# Autodesk Inventor assembly: 自動販賣機3.4
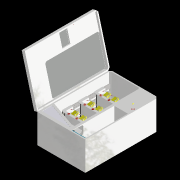
[picture p0: Inventor's stored thumbnail of the model, 180x180]
Saved by Autodesk Inventor 2020 (Build 240168000, 168)
## iProperties
Created: 2021-04-08
Part Number: 自動販賣機3.4
Document SubType Name: Assembly
Designer: 88690
Author: 88690
## Documents named in this file (33)
- C:\Users\88690\Desktop\自動販賣機\自動販賣機3.4.iam
- C:\Users\88690\Desktop\自動販賣機\上滑軌.ipt
- C:\Users\88690\Desktop\自動販賣機\上滑軌輪.ipt
- C:\Users\88690\Desktop\自動販賣機\下滑軌.ipt
- C:\Users\88690\Desktop\自動販賣機\下滑軌輪.ipt
- C:\Users\88690\Desktop\自動販賣機\本體.ipt
- C:\Users\88690\Desktop\自動販賣機\置物架.ipt
- C:\Users\88690\Desktop\自動販賣機\滾筒.ipt
- C:\Users\88690\Desktop\自動販賣機\蓋.ipt
- C:\Users\88690\Desktop\自動販賣機\鎖點支架.ipt
- C:\Users\88690\Desktop\自動販賣機\下支架右.ipt
- C:\Users\88690\Desktop\自動販賣機\上滑軌右.ipt
- C:\Users\88690\Desktop\自動販賣機\蝸桿支架.ipt
- C:\Users\88690\Desktop\自動販賣機\蝸桿滑塊.ipt
- C:\Users\88690\Desktop\自動販賣機\短蝸桿.ipt
- C:\Users\88690\Desktop\自動販賣機\長蝸桿.ipt
- C:\Users\88690\Desktop\自動販賣機\位移平台.ipt
- C:\Users\88690\Desktop\自動販賣機\取物窗.ipt
- C:\Users\88690\Desktop\自動販賣機\螺旋鉤子.ipt
- C:\Users\88690\Desktop\自動販賣機\螺旋鉤子底座.ipt
- C:\Users\88690\Desktop\自動販賣機\名牌1.ipt
- C:\Users\88690\Desktop\自動販賣機\名牌2.ipt
- C:\Users\88690\Desktop\自動販賣機\模擬商品.ipt
- C:\Users\88690\Desktop\自動販賣機\模擬錢幣.ipt
- C:\Users\88690\Desktop\自動販賣機\商品支架.ipt
- C:\Users\88690\Desktop\自動販賣機\名牌3.ipt
- C:\Users\88690\Desktop\自動販賣機\名牌4.ipt
- C:\Users\88690\Desktop\自動販賣機\名牌5.ipt
- C:\Users\88690\Desktop\自動販賣機\名牌6.ipt
- C:\Users\88690\Desktop\自動販賣機\名牌7.ipt
- C:\Users\88690\Desktop\自動販賣機\名牌8.ipt
- C:\Users\88690\Desktop\自動販賣機\名牌9.ipt
- C:\Users\88690\Desktop\自動販賣機\玻璃窗.ipt
## Components (110 placed, 32 different names)
1. 上滑軌:1 — 貼合:41, 貼合:42, 貼合:45, 相切:7, 貼合:183
2. 上滑軌輪:1 — 貼合:41, 貼合:42, 相切:1
3. 下滑軌:1 — 貼合:11, 貼合:12, 貼合:13, 貼合:15, 相切:1, 角度:40
4. 下滑軌輪:1 — 貼合:11, 貼合:12, 相切:7
5. 本體:1 — 齊平:1, 齊平:2, 齊平:3, 貼合:1, 貼合:2, 貼合:3, 貼合:4, 貼合:6, 貼合:7, 貼合:8, 貼合:9, 貼合:75, 貼合:76, 貼合:77, 貼合:78, 貼合:79, 貼合:80, 貼合:81, 貼合:82, 貼合:83, 貼合:84, 貼合:85, 貼合:86, 貼合:88, 貼合:89, 貼合:101, 齊平:23, 角度:1, 旋轉:1, 貼合:167, 角度:34, 貼合:169, 貼合:171, 貼合:172, 齊平:53, 齊平:58, 齊平:69
6. 置物架:1 — 貼合:45, 貼合:50, 貼合:51, 貼合:131, 貼合:143, 貼合:144, 貼合:145, 旋轉:3, 齊平:53, 角度:40, 貼合:183, 角度:41, 貼合:187, 相切:13, 相切:15, 貼合:227, 貼合:228, 貼合:229, 相切:16, 貼合:298, 貼合:299, 相切:17, 相切:18, 相切:19, 貼合:300, 貼合:301, 相切:20, 相切:21, 相切:22, 齊平:66, 齊平:67, 齊平:68, 貼合:448
7. 滾筒:1 — 貼合:75, 貼合:76, 齊平:14, 齊平:15, 齊平:16, 齊平:17, 齊平:18, 齊平:19, 齊平:20, 齊平:21, 齊平:22, 角度:12, 旋轉:1, 旋轉:1
8. 蓋:1 — 貼合:101, 齊平:23, 角度:1, 角度:2, 貼合:108, 貼合:164, 角度:34, 角度:35, 齊平:78, 貼合:455, 貼合:456
9. 鎖點支架:1 — 貼合:1, 貼合:2, 貼合:3, 齊平:4, 齊平:5, 齊平:6, 齊平:7, 貼合:5, 貼合:15
10. 鎖點支架:2 — 齊平:5, 齊平:7, 貼合:5, 貼合:13, 貼合:51
11. 鎖點支架:3 — 齊平:4, 齊平:6, 貼合:4
12. 鎖點支架:4 — 齊平:8, 齊平:10, 貼合:9
13. 鎖點支架:5 — 貼合:6, 貼合:7, 貼合:8, 齊平:8, 齊平:9, 齊平:10, 齊平:11, 貼合:10, 貼合:30
14. 鎖點支架:6 — 齊平:9, 齊平:11, 貼合:10, 貼合:28
15. 下支架右:1 — 貼合:26, 貼合:27, 貼合:28, 貼合:30, 相切:2, 貼合:74, 角度:41
16. 下滑軌輪:4 — 貼合:26, 貼合:27, 相切:10
17. 上滑軌右:1 — 貼合:46, 貼合:50, 相切:10, 貼合:186, 貼合:187
18. 上滑軌輪:2 — 貼合:46, 相切:2, 貼合:74, 貼合:186
19. 滾筒:2 — 齊平:14, 貼合:77, 旋轉:1, 旋轉:2, 角度:13
20. 滾筒:3 — 齊平:15, 貼合:78, 旋轉:2, 角度:14, 旋轉:3
21. 滾筒:4 — 齊平:16, 貼合:79, 角度:15, 旋轉:3, 旋轉:4
22. 滾筒:5 — 齊平:17, 貼合:80, 角度:16, 旋轉:4, 旋轉:5
23. 滾筒:6 — 齊平:18, 貼合:81, 角度:18, 旋轉:5, 旋轉:6
24. 滾筒:7 — 齊平:19, 貼合:82, 角度:19, 旋轉:6, 旋轉:7
25. 滾筒:8 — 齊平:20, 貼合:83, 角度:22, 旋轉:7, 旋轉:8
26. 滾筒:9 — 齊平:21, 貼合:84, 角度:20, 旋轉:8, 旋轉:9
27. 滾筒:10 — 齊平:22, 貼合:85, 角度:21, 旋轉:9
28. 蝸桿支架:1 — 貼合:86, 貼合:88, 貼合:89, 貼合:90, 貼合:91, 貼合:92, 貼合:93
29. 蝸桿滑塊:1 — 貼合:90, 貼合:91, 貼合:94, 貼合:95, 貼合:97, 貼合:98, 貼合:99
30. 短蝸桿:1 — 貼合:94, 貼合:95, 旋轉/轉換:1
31. 長蝸桿:1 — 貼合:92, 貼合:93, 角度:23, 旋轉/轉換:1
32. 位移平台:1 — 貼合:97, 貼合:98, 貼合:99, 貼合:167
33. 取物窗:1 — 角度:2, 貼合:108, 貼合:164, 角度:35
34. 螺旋鉤子:2 — 貼合:131, 角度:45, 貼合:221, 貼合:223, 貼合:230, 貼合:231, 貼合:232, 貼合:233
35. 螺旋鉤子底座:2 — 旋轉:3, 角度:44
36. 名牌1:1 — 貼合:143, 貼合:144, 角度:24, 齊平:30, 角度:25
37. 名牌2:1 — 貼合:145, 齊平:30, 角度:25, 齊平:71, 齊平:72, 角度:52
38. 模擬錢幣:1 — 貼合:169, 貼合:171, 貼合:172
39. 模擬商品:2 — 貼合:221, 相切:13, 貼合:230
40. 商品支架:1 — 貼合:227, 貼合:228, 貼合:229
41. 模擬商品:22 — 貼合:223, 相切:15, 貼合:231
42. 模擬商品:23 — 相切:16, 貼合:232, 貼合:233
43. 螺旋鉤子:3
44. 螺旋鉤子底座:3 — 貼合:298, 貼合:299
45. 模擬商品:24 — 相切:17
46. 模擬商品:25 — 相切:18
47. 模擬商品:26 — 相切:19
48. 螺旋鉤子:4
49. 螺旋鉤子底座:4 — 貼合:300, 貼合:301
50. 模擬商品:27 — 相切:20
51. 模擬商品:28 — 相切:21
52. 模擬商品:29 — 相切:22
53. 上滑軌:2 — 齊平:57
54. 上滑軌輪:3 — 貼合:398
55. 下滑軌:2 — 齊平:60, 貼合:398
56. 下滑軌輪:5
57. 置物架:2 — 齊平:56, 齊平:58, 齊平:59, 齊平:60, 齊平:66, 齊平:67, 齊平:70, 貼合:449, 貼合:450, 貼合:451
58. 下支架右:2 — 齊平:59
59. 下滑軌輪:6
60. 上滑軌右:2 — 齊平:56, 齊平:57
61. 上滑軌輪:4
62. 螺旋鉤子:5
63. 螺旋鉤子底座:5
64. 模擬商品:30
65. 商品支架:2
66. 模擬商品:31
67. 模擬商品:32
68. 螺旋鉤子:6
69. 螺旋鉤子底座:6
70. 模擬商品:33
71. 模擬商品:34
72. 模擬商品:35
73. 螺旋鉤子:7
74. 螺旋鉤子底座:7
75. 模擬商品:36
76. 模擬商品:37
77. 模擬商品:38
78. 上滑軌:3
79. 上滑軌輪:5
80. 下滑軌:3
81. 下滑軌輪:7
82. 置物架:3 — 齊平:68, 齊平:69, 齊平:70, 貼合:452, 貼合:453, 貼合:454
83. 下支架右:3
84. 下滑軌輪:8
85. 上滑軌右:3
86. 上滑軌輪:6
87. 螺旋鉤子:8
88. 螺旋鉤子底座:8
89. 模擬商品:39
90. 商品支架:3
91. 模擬商品:40
92. 模擬商品:41
93. 螺旋鉤子:9
94. 螺旋鉤子底座:9
95. 模擬商品:42
96. 模擬商品:43
97. 模擬商品:44
98. 螺旋鉤子:10
99. 螺旋鉤子底座:10
100. 模擬商品:45
101. 模擬商品:46
102. 模擬商品:47
103. 名牌3:1 — 貼合:448, 齊平:71, 角度:52, 角度:53
104. 名牌4:1 — 貼合:449, 齊平:72, 齊平:73, 角度:53, 角度:54
105. 名牌5:1 — 貼合:450, 齊平:73, 齊平:74, 角度:54, 角度:55
106. 名牌6:1 — 貼合:451, 齊平:74, 齊平:75, 角度:55, 角度:56
107. 名牌7:1 — 貼合:452, 齊平:77, 角度:56, 角度:57
108. 名牌8:1 — 貼合:453, 齊平:76, 齊平:77, 角度:57, 角度:58
109. 名牌9:1 — 貼合:454, 齊平:75, 齊平:76, 角度:58
110. 玻璃窗:1 — 齊平:78, 貼合:455, 貼合:456
## Relationships (324: Mate 194, Flush 45, Tangent 39, Angle 32, RelateRotation 9, RevoluteJoint 4, RelateRotateTranslate 1)
- 齊平:1 [Flush]: 本體:1
- 齊平:2 [Flush]: 本體:1
- 齊平:3 [Flush]: 本體:1
- 貼合:1 [Mate] (180 mm): 本體:1 ↔ 鎖點支架:1
- 貼合:2 [Mate]: 本體:1 ↔ 鎖點支架:1
- 貼合:3 [Mate]: 本體:1 ↔ 鎖點支架:1
- 齊平:4 [Flush]: 鎖點支架:1 ↔ 鎖點支架:3
- 齊平:5 [Flush]: 鎖點支架:1 ↔ 鎖點支架:2
- 齊平:6 [Flush]: 鎖點支架:1 ↔ 鎖點支架:3
- 齊平:7 [Flush]: 鎖點支架:1 ↔ 鎖點支架:2
- 貼合:4 [Mate]: 本體:1 ↔ 鎖點支架:3
- 貼合:5 [Mate] (55 mm): 鎖點支架:1 ↔ 鎖點支架:2
- 貼合:6 [Mate]: 本體:1 ↔ 鎖點支架:5
- 貼合:7 [Mate]: 本體:1 ↔ 鎖點支架:5
- 貼合:8 [Mate] (180 mm): 本體:1 ↔ 鎖點支架:5
- 齊平:8 [Flush]: 鎖點支架:4 ↔ 鎖點支架:5
- 齊平:9 [Flush]: 鎖點支架:5 ↔ 鎖點支架:6
- 齊平:10 [Flush]: 鎖點支架:4 ↔ 鎖點支架:5
- 齊平:11 [Flush]: 鎖點支架:5 ↔ 鎖點支架:6
- 貼合:9 [Mate]: 本體:1 ↔ 鎖點支架:4
- 貼合:10 [Mate] (55 mm): 鎖點支架:5 ↔ 鎖點支架:6
- 貼合:11 [Mate]: 下滑軌:1 ↔ 下滑軌輪:1
- 貼合:12 [Mate]: 下滑軌:1 ↔ 下滑軌輪:1
- 貼合:13 [Mate]: 下滑軌:1 ↔ 鎖點支架:2
- 貼合:15 [Mate]: 下滑軌:1 ↔ 鎖點支架:1
- 貼合:26 [Mate]: 下支架右:1 ↔ 下滑軌輪:4
- 貼合:27 [Mate]: 下支架右:1 ↔ 下滑軌輪:4
- 貼合:28 [Mate]: 鎖點支架:6 ↔ 下支架右:1
- 貼合:30 [Mate]: 鎖點支架:5 ↔ 下支架右:1
- 貼合:41 [Mate]: 上滑軌:1 ↔ 上滑軌輪:1
- 貼合:42 [Mate]: 上滑軌:1 ↔ 上滑軌輪:1
- 貼合:45 [Mate]: 上滑軌:1 ↔ 置物架:1
- 貼合:46 [Mate]: 上滑軌右:1 ↔ 上滑軌輪:2
- 貼合:50 [Mate]: 置物架:1 ↔ 上滑軌右:1
- 相切:1 [Tangent]: 上滑軌輪:1 ↔ 下滑軌:1
- 相切:2 [Tangent]: 下支架右:1 ↔ 上滑軌輪:2
- 貼合:51 [Mate]: 置物架:1 ↔ 鎖點支架:2
- 貼合:74 [Mate]: 下支架右:1 ↔ 上滑軌輪:2
- 貼合:75 [Mate]: 本體:1 ↔ 滾筒:1
- 貼合:76 [Mate]: 本體:1 ↔ 滾筒:1
- 齊平:14 [Flush]: 滾筒:1 ↔ 滾筒:2
- 齊平:15 [Flush]: 滾筒:1 ↔ 滾筒:3
- 齊平:16 [Flush]: 滾筒:1 ↔ 滾筒:4
- 齊平:17 [Flush]: 滾筒:1 ↔ 滾筒:5
- 齊平:18 [Flush]: 滾筒:1 ↔ 滾筒:6
- 齊平:19 [Flush]: 滾筒:1 ↔ 滾筒:7
- 齊平:20 [Flush]: 滾筒:1 ↔ 滾筒:8
- 齊平:21 [Flush]: 滾筒:1 ↔ 滾筒:9
- 齊平:22 [Flush]: 滾筒:1 ↔ 滾筒:10
- 貼合:77 [Mate]: 本體:1 ↔ 滾筒:2
- 貼合:78 [Mate]: 本體:1 ↔ 滾筒:3
- 貼合:79 [Mate]: 本體:1 ↔ 滾筒:4
- 貼合:80 [Mate]: 本體:1 ↔ 滾筒:5
- 貼合:81 [Mate]: 本體:1 ↔ 滾筒:6
- 貼合:82 [Mate]: 本體:1 ↔ 滾筒:7
- 貼合:83 [Mate]: 本體:1 ↔ 滾筒:8
- 貼合:84 [Mate]: 本體:1 ↔ 滾筒:9
- 貼合:85 [Mate]: 本體:1 ↔ 滾筒:10
- 貼合:86 [Mate]: 本體:1 ↔ 蝸桿支架:1
- 貼合:88 [Mate]: 本體:1 ↔ 蝸桿支架:1
- 貼合:89 [Mate]: 本體:1 ↔ 蝸桿支架:1
- 貼合:90 [Mate]: 蝸桿支架:1 ↔ 蝸桿滑塊:1
- 貼合:91 [Mate]: 蝸桿支架:1 ↔ 蝸桿滑塊:1
- 貼合:92 [Mate]: 蝸桿支架:1 ↔ 長蝸桿:1
- 貼合:93 [Mate]: 蝸桿支架:1 ↔ 長蝸桿:1
- 貼合:94 [Mate]: 蝸桿滑塊:1 ↔ 短蝸桿:1
- 貼合:95 [Mate]: 蝸桿滑塊:1 ↔ 短蝸桿:1
- 貼合:97 [Mate]: 蝸桿滑塊:1 ↔ 位移平台:1
- 貼合:98 [Mate]: 蝸桿滑塊:1 ↔ 位移平台:1
- 貼合:99 [Mate]: 蝸桿滑塊:1 ↔ 位移平台:1
- 貼合:101 [Mate]: 本體:1 ↔ 蓋:1
- 齊平:23 [Flush]: 本體:1 ↔ 蓋:1
- 角度:1 [Angle] (45 deg): 本體:1 ↔ 蓋:1
- 角度:2 [Angle] (180 deg): 蓋:1 ↔ 取物窗:1
- 貼合:108 [Mate]: 蓋:1 ↔ 取物窗:1
- [Mate]: 螺旋鉤子:2 ↔ 螺旋鉤子底座:2
- [Mate]: 螺旋鉤子:2 ↔ 螺旋鉤子底座:2
- 貼合:131 [Mate]: 置物架:1 ↔ 螺旋鉤子:2
- 角度:12 [Angle] (4455 deg): 滾筒:1
- 旋轉:1 [RelateRotation] (1 ul): 滾筒:1 ↔ 滾筒:2
- 旋轉:2 [RelateRotation] (1 ul): 滾筒:2 ↔ 滾筒:3
- 角度:13 [Angle] (135 deg): 滾筒:2
- 角度:14 [Angle] (135 deg): 滾筒:3
- 角度:15 [Angle] (135 deg): 滾筒:4
- 角度:16 [Angle] (135 deg): 滾筒:5
- 角度:18 [Angle] (135 deg): 滾筒:6
- 角度:19 [Angle] (135 deg): 滾筒:7
- 角度:20 [Angle] (135 deg): 滾筒:9
- 角度:21 [Angle] (135 deg): 滾筒:10
- 角度:22 [Angle] (135 deg): 滾筒:8
- 旋轉:3 [RelateRotation] (1 ul): 滾筒:3 ↔ 滾筒:4
- 旋轉:4 [RelateRotation] (1 ul): 滾筒:4 ↔ 滾筒:5
- 旋轉:5 [RelateRotation] (1 ul): 滾筒:5 ↔ 滾筒:6
- 旋轉:6 [RelateRotation] (1 ul): 滾筒:6 ↔ 滾筒:7
- 旋轉:7 [RelateRotation] (1 ul): 滾筒:7 ↔ 滾筒:8
- 旋轉:8 [RelateRotation] (1 ul): 滾筒:8 ↔ 滾筒:9
- 旋轉:9 [RelateRotation] (1 ul): 滾筒:9 ↔ 滾筒:10
- 旋轉:1 [RevoluteJoint]: 本體:1 ↔ 滾筒:1
- 角度:23 [Angle] (0 deg): 長蝸桿:1
- 旋轉/轉換:1 [RelateRotateTranslate] (103.673 mm): 短蝸桿:1 ↔ 長蝸桿:1
- 貼合:143 [Mate]: 置物架:1 ↔ 名牌1:1
- 貼合:144 [Mate]: 置物架:1 ↔ 名牌1:1
- 角度:24 [Angle] (0 deg): 名牌1:1
- 貼合:145 [Mate]: 置物架:1 ↔ 名牌2:1
- 齊平:30 [Flush]: 名牌1:1 ↔ 名牌2:1
- 角度:25 [Angle] (0 deg): 名牌1:1 ↔ 名牌2:1
- 旋轉:3 [RevoluteJoint]: 置物架:1 ↔ 螺旋鉤子底座:2
- 貼合:164 [Mate]: 蓋:1 ↔ 取物窗:1
- 貼合:167 [Mate]: 本體:1 ↔ 位移平台:1
- 角度:34 [Angle] (75 deg): 本體:1 ↔ 蓋:1
- 角度:35 [Angle] (180 deg): 蓋:1 ↔ 取物窗:1
- 貼合:169 [Mate] (0.5 mm): 本體:1 ↔ 模擬錢幣:1
- 貼合:171 [Mate]: 本體:1 ↔ 模擬錢幣:1
- 貼合:172 [Mate] (150 mm): 本體:1 ↔ 模擬錢幣:1
- 齊平:53 [Flush] (-390 mm): 本體:1 ↔ 置物架:1
- 角度:40 [Angle] (0 deg): 下滑軌:1 ↔ 置物架:1
- 相切:7 [Tangent]: 上滑軌:1 ↔ 下滑軌輪:1
- 貼合:183 [Mate]: 上滑軌:1 ↔ 置物架:1
- 角度:41 [Angle] (0 deg): 置物架:1 ↔ 下支架右:1
- 相切:10 [Tangent]: 下滑軌輪:4 ↔ 上滑軌右:1
- 貼合:186 [Mate]: 上滑軌右:1 ↔ 上滑軌輪:2
- 貼合:187 [Mate]: 置物架:1 ↔ 上滑軌右:1
- 角度:44 [Angle] (0 deg): 螺旋鉤子底座:2
- 角度:45 [Angle] (180 deg): 螺旋鉤子:2
- 貼合:221 [Mate]: 螺旋鉤子:2 ↔ 模擬商品:2
- 相切:13 [Tangent]: 置物架:1 ↔ 模擬商品:2
- 貼合:223 [Mate]: 螺旋鉤子:2 ↔ 模擬商品:22
- 相切:15 [Tangent]: 置物架:1 ↔ 模擬商品:22
- 貼合:227 [Mate]: 置物架:1 ↔ 商品支架:1
- 貼合:228 [Mate]: 置物架:1 ↔ 商品支架:1
- 貼合:229 [Mate]: 置物架:1 ↔ 商品支架:1
- 貼合:230 [Mate]: 螺旋鉤子:2 ↔ 模擬商品:2
- 貼合:231 [Mate]: 螺旋鉤子:2 ↔ 模擬商品:22
- 相切:16 [Tangent]: 置物架:1 ↔ 模擬商品:23
- 貼合:232 [Mate]: 螺旋鉤子:2 ↔ 模擬商品:23
- 貼合:233 [Mate]: 螺旋鉤子:2 ↔ 模擬商品:23
- [Mate]: 螺旋鉤子:3 ↔ 螺旋鉤子底座:3
- [Mate]: 螺旋鉤子:3 ↔ 螺旋鉤子底座:3
- [Mate]: 螺旋鉤子:3 ↔ 模擬商品:24
- [Mate]: 螺旋鉤子:3 ↔ 模擬商品:25
- [Mate]: 螺旋鉤子:3 ↔ 模擬商品:24
- [Mate]: 螺旋鉤子:3 ↔ 模擬商品:25
- [Mate]: 螺旋鉤子:3 ↔ 模擬商品:26
- [Mate]: 螺旋鉤子:3 ↔ 模擬商品:26
- [Mate]: 螺旋鉤子:4 ↔ 螺旋鉤子底座:4
- [Mate]: 螺旋鉤子:4 ↔ 螺旋鉤子底座:4
- [Mate]: 螺旋鉤子:4 ↔ 模擬商品:27
- [Mate]: 螺旋鉤子:4 ↔ 模擬商品:28
- [Mate]: 螺旋鉤子:4 ↔ 模擬商品:27
- [Mate]: 螺旋鉤子:4 ↔ 模擬商品:28
- [Mate]: 螺旋鉤子:4 ↔ 模擬商品:29
- [Mate]: 螺旋鉤子:4 ↔ 模擬商品:29
- 貼合:298 [Mate]: 置物架:1 ↔ 螺旋鉤子底座:3
- 貼合:299 [Mate]: 置物架:1 ↔ 螺旋鉤子底座:3
- 相切:17 [Tangent]: 置物架:1 ↔ 模擬商品:24
- 相切:18 [Tangent]: 置物架:1 ↔ 模擬商品:25
- 相切:19 [Tangent]: 置物架:1 ↔ 模擬商品:26
- 貼合:300 [Mate]: 置物架:1 ↔ 螺旋鉤子底座:4
- 貼合:301 [Mate]: 置物架:1 ↔ 螺旋鉤子底座:4
- 相切:20 [Tangent]: 置物架:1 ↔ 模擬商品:27
- 相切:21 [Tangent]: 置物架:1 ↔ 模擬商品:28
- 相切:22 [Tangent]: 置物架:1 ↔ 模擬商品:29
- [Mate]: 下滑軌:2 ↔ 下滑軌輪:5
- [Mate]: 下滑軌:2 ↔ 下滑軌輪:5
- [Mate]: 下支架右:2 ↔ 下滑軌輪:6
- [Mate]: 下支架右:2 ↔ 下滑軌輪:6
- [Mate]: 上滑軌:2 ↔ 上滑軌輪:3
- [Mate]: 上滑軌:2 ↔ 上滑軌輪:3
- [Mate]: 上滑軌:2 ↔ 置物架:2
- [Mate]: 上滑軌右:2 ↔ 上滑軌輪:4
- [Mate]: 置物架:2 ↔ 上滑軌右:2
- [Tangent]: 上滑軌輪:3 ↔ 下滑軌:2
- [Tangent]: 下支架右:2 ↔ 上滑軌輪:4
- [Mate]: 下支架右:2 ↔ 上滑軌輪:4
- [Mate]: 螺旋鉤子:5 ↔ 螺旋鉤子底座:5
- [Mate]: 螺旋鉤子:5 ↔ 螺旋鉤子底座:5
- [Mate]: 置物架:2 ↔ 螺旋鉤子:5
- [RevoluteJoint]: 置物架:2 ↔ 螺旋鉤子底座:5
- [Angle] (0 deg): 下滑軌:2 ↔ 置物架:2
- [Tangent]: 上滑軌:2 ↔ 下滑軌輪:5
- [Mate]: 上滑軌:2 ↔ 置物架:2
- [Angle] (0 deg): 置物架:2 ↔ 下支架右:2
- [Tangent]: 下滑軌輪:6 ↔ 上滑軌右:2
- [Mate]: 上滑軌右:2 ↔ 上滑軌輪:4
- [Mate]: 置物架:2 ↔ 上滑軌右:2
- [Mate]: 螺旋鉤子:5 ↔ 模擬商品:30
- [Tangent]: 置物架:2 ↔ 模擬商品:30
- [Mate]: 螺旋鉤子:5 ↔ 模擬商品:31
- [Tangent]: 置物架:2 ↔ 模擬商品:31
- [Mate]: 置物架:2 ↔ 商品支架:2
- [Mate]: 置物架:2 ↔ 商品支架:2
- [Mate]: 置物架:2 ↔ 商品支架:2
- [Mate]: 螺旋鉤子:5 ↔ 模擬商品:30
- [Mate]: 螺旋鉤子:5 ↔ 模擬商品:31
- [Tangent]: 置物架:2 ↔ 模擬商品:32
- [Mate]: 螺旋鉤子:5 ↔ 模擬商品:32
- [Mate]: 螺旋鉤子:5 ↔ 模擬商品:32
- [Mate]: 螺旋鉤子:6 ↔ 螺旋鉤子底座:6
- [Mate]: 螺旋鉤子:6 ↔ 螺旋鉤子底座:6
- [Mate]: 螺旋鉤子:6 ↔ 模擬商品:33
- [Mate]: 螺旋鉤子:6 ↔ 模擬商品:34
- [Mate]: 螺旋鉤子:6 ↔ 模擬商品:33
- [Mate]: 螺旋鉤子:6 ↔ 模擬商品:34
- [Mate]: 螺旋鉤子:6 ↔ 模擬商品:35
- [Mate]: 螺旋鉤子:6 ↔ 模擬商品:35
- [Mate]: 螺旋鉤子:7 ↔ 螺旋鉤子底座:7
- [Mate]: 螺旋鉤子:7 ↔ 螺旋鉤子底座:7
- [Mate]: 螺旋鉤子:7 ↔ 模擬商品:36
- [Mate]: 螺旋鉤子:7 ↔ 模擬商品:37
- [Mate]: 螺旋鉤子:7 ↔ 模擬商品:36
- [Mate]: 螺旋鉤子:7 ↔ 模擬商品:37
- [Mate]: 螺旋鉤子:7 ↔ 模擬商品:38
- [Mate]: 螺旋鉤子:7 ↔ 模擬商品:38
- [Mate]: 置物架:2 ↔ 螺旋鉤子底座:6
- [Mate]: 置物架:2 ↔ 螺旋鉤子底座:6
- [Tangent]: 置物架:2 ↔ 模擬商品:33
- [Tangent]: 置物架:2 ↔ 模擬商品:34
- [Tangent]: 置物架:2 ↔ 模擬商品:35
- [Mate]: 置物架:2 ↔ 螺旋鉤子底座:7
- [Mate]: 置物架:2 ↔ 螺旋鉤子底座:7
- [Tangent]: 置物架:2 ↔ 模擬商品:36
- [Tangent]: 置物架:2 ↔ 模擬商品:37
- [Tangent]: 置物架:2 ↔ 模擬商品:38
- 齊平:56 [Flush] (135 mm): 置物架:2 ↔ 上滑軌右:2
- 齊平:57 [Flush]: 上滑軌:2 ↔ 上滑軌右:2
- 齊平:58 [Flush]: 本體:1 ↔ 置物架:2
- 齊平:59 [Flush]: 置物架:2 ↔ 下支架右:2
- 齊平:60 [Flush]: 下滑軌:2 ↔ 置物架:2
- 貼合:398 [Mate]: 上滑軌輪:3 ↔ 下滑軌:2
- [Mate]: 下滑軌:3 ↔ 下滑軌輪:7
- [Mate]: 下滑軌:3 ↔ 下滑軌輪:7
- [Mate]: 下支架右:3 ↔ 下滑軌輪:8
- [Mate]: 下支架右:3 ↔ 下滑軌輪:8
- [Mate]: 上滑軌:3 ↔ 上滑軌輪:5
- [Mate]: 上滑軌:3 ↔ 上滑軌輪:5
- [Mate]: 上滑軌:3 ↔ 置物架:3
- [Mate]: 上滑軌右:3 ↔ 上滑軌輪:6
- [Mate]: 置物架:3 ↔ 上滑軌右:3
- [Tangent]: 上滑軌輪:5 ↔ 下滑軌:3
- [Tangent]: 下支架右:3 ↔ 上滑軌輪:6
- [Mate]: 下支架右:3 ↔ 上滑軌輪:6
- [Mate]: 螺旋鉤子:8 ↔ 螺旋鉤子底座:8
- [Mate]: 螺旋鉤子:8 ↔ 螺旋鉤子底座:8
- [Mate]: 置物架:3 ↔ 螺旋鉤子:8
- [RevoluteJoint]: 置物架:3 ↔ 螺旋鉤子底座:8
- [Angle] (0 deg): 下滑軌:3 ↔ 置物架:3
- [Tangent]: 上滑軌:3 ↔ 下滑軌輪:7
- [Mate]: 上滑軌:3 ↔ 置物架:3
- [Angle] (0 deg): 置物架:3 ↔ 下支架右:3
- [Tangent]: 下滑軌輪:8 ↔ 上滑軌右:3
- [Mate]: 上滑軌右:3 ↔ 上滑軌輪:6
- [Mate]: 置物架:3 ↔ 上滑軌右:3
- [Mate]: 螺旋鉤子:8 ↔ 模擬商品:39
- [Tangent]: 置物架:3 ↔ 模擬商品:39
- [Mate]: 螺旋鉤子:8 ↔ 模擬商品:40
- [Tangent]: 置物架:3 ↔ 模擬商品:40
- [Mate]: 置物架:3 ↔ 商品支架:3
- [Mate]: 置物架:3 ↔ 商品支架:3
- [Mate]: 置物架:3 ↔ 商品支架:3
- [Mate]: 螺旋鉤子:8 ↔ 模擬商品:39
- [Mate]: 螺旋鉤子:8 ↔ 模擬商品:40
- [Tangent]: 置物架:3 ↔ 模擬商品:41
- [Mate]: 螺旋鉤子:8 ↔ 模擬商品:41
- [Mate]: 螺旋鉤子:8 ↔ 模擬商品:41
- [Mate]: 螺旋鉤子:9 ↔ 螺旋鉤子底座:9
- [Mate]: 螺旋鉤子:9 ↔ 螺旋鉤子底座:9
- [Mate]: 螺旋鉤子:9 ↔ 模擬商品:42
- [Mate]: 螺旋鉤子:9 ↔ 模擬商品:43
- [Mate]: 螺旋鉤子:9 ↔ 模擬商品:42
- [Mate]: 螺旋鉤子:9 ↔ 模擬商品:43
- [Mate]: 螺旋鉤子:9 ↔ 模擬商品:44
- [Mate]: 螺旋鉤子:9 ↔ 模擬商品:44
- [Mate]: 螺旋鉤子:10 ↔ 螺旋鉤子底座:10
- [Mate]: 螺旋鉤子:10 ↔ 螺旋鉤子底座:10
- [Mate]: 螺旋鉤子:10 ↔ 模擬商品:45
- [Mate]: 螺旋鉤子:10 ↔ 模擬商品:46
- [Mate]: 螺旋鉤子:10 ↔ 模擬商品:45
- [Mate]: 螺旋鉤子:10 ↔ 模擬商品:46
- [Mate]: 螺旋鉤子:10 ↔ 模擬商品:47
- [Mate]: 螺旋鉤子:10 ↔ 模擬商品:47
- [Mate]: 置物架:3 ↔ 螺旋鉤子底座:9
- [Mate]: 置物架:3 ↔ 螺旋鉤子底座:9
- [Tangent]: 置物架:3 ↔ 模擬商品:42
- [Tangent]: 置物架:3 ↔ 模擬商品:43
- [Tangent]: 置物架:3 ↔ 模擬商品:44
- [Mate]: 置物架:3 ↔ 螺旋鉤子底座:10
- [Mate]: 置物架:3 ↔ 螺旋鉤子底座:10
- [Tangent]: 置物架:3 ↔ 模擬商品:45
- [Tangent]: 置物架:3 ↔ 模擬商品:46
- [Tangent]: 置物架:3 ↔ 模擬商品:47
- [Flush] (135 mm): 置物架:3 ↔ 上滑軌右:3
- [Flush]: 上滑軌:3 ↔ 上滑軌右:3
- [Flush]: 置物架:3 ↔ 下支架右:3
- [Flush]: 下滑軌:3 ↔ 置物架:3
- [Mate]: 上滑軌輪:5 ↔ 下滑軌:3
- 齊平:66 [Flush]: 置物架:1 ↔ 置物架:2
- 齊平:67 [Flush]: 置物架:1 ↔ 置物架:2
- 齊平:68 [Flush]: 置物架:1 ↔ 置物架:3
- 齊平:69 [Flush]: 本體:1 ↔ 置物架:3
- 齊平:70 [Flush]: 置物架:2 ↔ 置物架:3
- 貼合:448 [Mate]: 置物架:1 ↔ 名牌3:1
- 齊平:71 [Flush]: 名牌2:1 ↔ 名牌3:1
- 貼合:449 [Mate]: 置物架:2 ↔ 名牌4:1
- 貼合:450 [Mate]: 置物架:2 ↔ 名牌5:1
- 貼合:451 [Mate]: 置物架:2 ↔ 名牌6:1
- 貼合:452 [Mate]: 置物架:3 ↔ 名牌7:1
- 貼合:453 [Mate]: 置物架:3 ↔ 名牌8:1
- 貼合:454 [Mate]: 置物架:3 ↔ 名牌9:1
- 齊平:72 [Flush]: 名牌2:1 ↔ 名牌4:1
- 齊平:73 [Flush]: 名牌4:1 ↔ 名牌5:1
- 齊平:74 [Flush]: 名牌5:1 ↔ 名牌6:1
- 齊平:75 [Flush]: 名牌6:1 ↔ 名牌9:1
- 齊平:76 [Flush]: 名牌8:1 ↔ 名牌9:1
- 齊平:77 [Flush]: 名牌7:1 ↔ 名牌8:1
- 角度:52 [Angle] (0 deg): 名牌2:1 ↔ 名牌3:1
- 角度:53 [Angle] (0 deg): 名牌3:1 ↔ 名牌4:1
- 角度:54 [Angle] (0 deg): 名牌4:1 ↔ 名牌5:1
- 角度:55 [Angle] (0 deg): 名牌5:1 ↔ 名牌6:1
- 角度:56 [Angle] (0 deg): 名牌6:1 ↔ 名牌7:1
- 角度:57 [Angle] (0 deg): 名牌7:1 ↔ 名牌8:1
- 角度:58 [Angle] (0 deg): 名牌8:1 ↔ 名牌9:1
- 齊平:78 [Flush]: 蓋:1 ↔ 玻璃窗:1
- 貼合:455 [Mate]: 蓋:1 ↔ 玻璃窗:1
- 貼合:456 [Mate]: 蓋:1 ↔ 玻璃窗:1
## Named parameters: d158_d154 = 0 mm, d159_d155 = 0 mm, d589_d572 = 0 mm, d590_d575 = 0 mm, d591_d584 = 0 mm, d592_d585 = 0 mm, d593_d587 = 0 mm, d594_d588 = 0 mm, d595_d158_d154 = 0 mm, d596_d159_d155 = 0 mm, d597_d572 = 0 mm, d598_d575 = 0 mm, d599_d584 = 0 mm, d600_d585 = 0 mm, d601_d587 = 0 mm, d602_d588 = 0 mm, d603_d158_d154 = 0 mm, d604_d159_d155 = 0 mm, d663_d653 = 0 mm, d664_d654 = 0 mm, d665_d655 = 0 mm, d666_d656 = 0 mm, d667_d657 = 0 mm, d668_d658 = 0 mm, d669_d659 = 0 mm, d670_d660 = 0 mm, d671_d661 = 0 mm, d672_d662 = 0 mm, d673_d458 = 0 deg, d674_d459 = 0 mm, d675_d460 = 0 mm, d676_d461 = 0 mm, d677_d572 = 0 mm, d678_d573 = 0 mm, d679_d575 = 0 mm, d680_d580 = 0 mm, d681_d581 = 0 mm, d682_d582 = 0 mm, d683_d583 = 0 mm, d684_d584 = 0 mm, d685_d585 = 0 mm, d686_d586 = 0 mm, d687_d587 = 0 mm, d688_d588 = 0 mm, d689_d589_d572 = 0 mm, d690_d590_d575 = 0 mm, d691_d591_d584 = 0 mm, d692_d592_d585 = 0 mm, d693_d593_d587 = 0 mm, d694_d594_d588 = 0 mm, d695_d595_d158_d154 = 0 mm, d696_d596_d159_d155 = 0 mm, d697_d597_d572 = 0 mm, d698_d598_d575 = 0 mm, d699_d599_d584 = 0 mm, d700_d600_d585 = 0 mm, d701_d601_d587 = 0 mm, d702_d602_d588 = 0 mm, d703_d603_d158_d154 = 0 mm, d704_d604_d159_d155 = 0 mm, d705_d451 = 0 deg, d706_d452 = 0 mm, d707_d453 = 0 mm, d708_d298 = 0 mm, d709_d299 = 90 deg, d715_d158_d154 = 0 mm, d716_d159_d155 = 0 mm, d717_d181 = 0 mm, d718_d64 = 0 mm, d719_d94 = 0 mm, d720_d21 = 0 mm, d721_d22 = 0 mm, d722_d37 = 0 mm, d723_d38 = 0 mm, d724_d52 = 0 mm, d725_d53 = 0 mm, d726_d56 = 0 mm, d727_d58 = 0 mm, d728_d62 = 0 mm, d729_d63 = 0 mm, d816_d809 = 135 mm, d817_d810 = 0 mm, d818_d812 = 0 mm, d819_d813 = 0 mm, d820_d814 = 0 mm, d821_d663_d653 = 0 mm, d822_d664_d654 = 0 mm, d823_d665_d655 = 0 mm, d824_d666_d656 = 0 mm, d825_d667_d657 = 0 mm, d826_d668_d658 = 0 mm, d827_d669_d659 = 0 mm, d828_d670_d660 = 0 mm, d829_d671_d661 = 0 mm, d830_d672_d662 = 0 mm, d831_d673_d458 = 0 deg, d832_d674_d459 = 0 mm, d833_d675_d460 = 0 mm, d834_d676_d461 = 0 mm, d835_d677_d572 = 0 mm, d836_d678_d573 = 0 mm, d837_d679_d575 = 0 mm, d838_d680_d580 = 0 mm, d839_d681_d581 = 0 mm, d840_d682_d582 = 0 mm, d841_d683_d583 = 0 mm, d842_d684_d584 = 0 mm, d843_d685_d585 = 0 mm, d844_d686_d586 = 0 mm, d845_d687_d587 = 0 mm, d846_d688_d588 = 0 mm, d847_d689_d589_d572 = 0 mm, d848_d690_d590_d575 = 0 mm, d849_d691_d591_d584 = 0 mm, d850_d692_d592_d585 = 0 mm, d851_d693_d593_d587 = 0 mm, d852_d694_d594_d588 = 0 mm, d853_d695_d595_d158_d154 = 0 mm, d854_d696_d596_d159_d155 = 0 mm, d855_d697_d597_d572 = 0 mm, d856_d698_d598_d575 = 0 mm, d857_d699_d599_d584 = 0 mm, d858_d700_d600_d585 = 0 mm, d859_d701_d601_d587 = 0 mm, d860_d702_d602_d588 = 0 mm, d861_d703_d603_d158_d154 = 0 mm, d862_d704_d604_d159_d155 = 0 mm, d863_d705_d451 = 0 deg, d864_d706_d452 = 0 mm, d865_d707_d453 = 0 mm, d866_d708_d298 = 0 mm, d867_d709_d299 = 90 deg, d873_d715_d158_d154 = 0 mm, d874_d716_d159_d155 = 0 mm, d875_d717_d181 = 0 mm, d876_d718_d64 = 0 mm, d877_d719_d94 = 0 mm, d878_d720_d21 = 0 mm, d879_d721_d22 = 0 mm, d880_d722_d37 = 0 mm, d881_d723_d38 = 0 mm, d882_d724_d52 = 0 mm, d883_d725_d53 = 0 mm, d884_d726_d56 = 0 mm, d885_d727_d58 = 0 mm, d886_d728_d62 = 0 mm, d887_d729_d63 = 0 mm
